# Autodesk Inventor assembly: Rotation Resistor Assembly
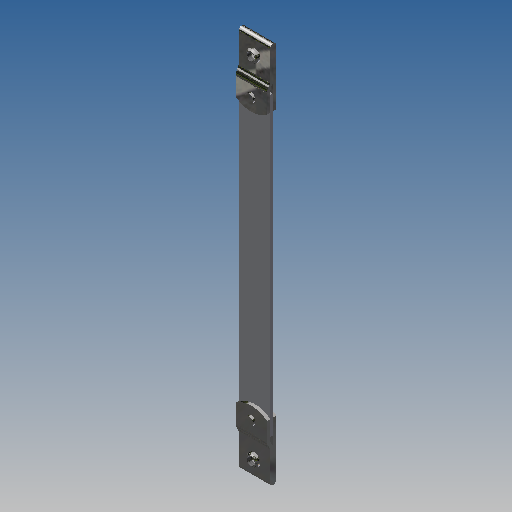
[picture p0: Inventor's stored thumbnail of the model, 512x512]
Saved by Autodesk Inventor 2018 (Build 220112000, 112)
## iProperties
Created: 2018-02-27
Part Number: Rotation Resistor Assembly
Document SubType Name: Assembly
Designer: 232963
Author: 232963
## Documents named in this file (4)
- D:\Cole\Documents\GitHub\SchoolCAD\ReverseEngineering\Rotation Resistor Assembly.iam
- D:\Cole\Documents\GitHub\SchoolCAD\ReverseEngineering\Rotation Resistor-01.ipt
- D:\Cole\Documents\GitHub\SchoolCAD\ReverseEngineering\Rivet.ipt
- D:\Cole\Documents\GitHub\SchoolCAD\ReverseEngineering\End Resistor Peice.ipt
## Components (5 placed, 3 different names)
1. Rotation Resistor-01:1 — Flush:1, Flush:2
2. Rivet:1 — Insert:1
3. Rivet:2 — Insert:2
4. End Resistor Peice:1 — Insert:1, Flush:1
5. End Resistor Peice:2 — Flush:2, Insert:2
## Relationships (4: Insert 2, Flush 2)
- Insert:1: Rivet:1 ↔ End Resistor Peice:1
- Flush:1: Rotation Resistor-01:1 ↔ End Resistor Peice:1
- Flush:2: Rotation Resistor-01:1 ↔ End Resistor Peice:2
- Insert:2: Rivet:2 ↔ End Resistor Peice:2
